# Autodesk Inventor assembly: Assembly1
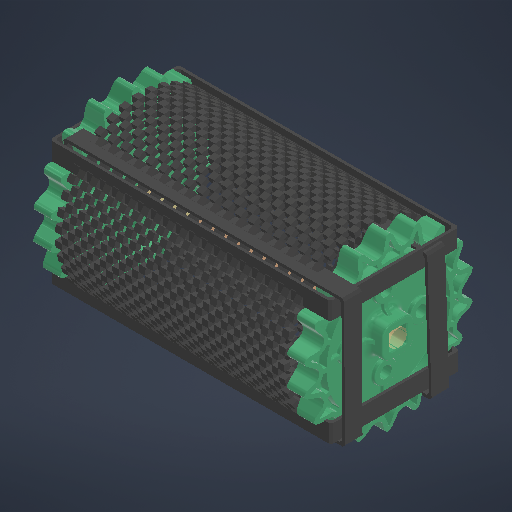
[picture p0: Inventor's stored thumbnail of the model, 512x512]
Saved by Autodesk Inventor 2025.2 (Build 292293000, 293)
## iProperties
Created: 2026-01-02
Part Number: Assembly1
Document SubType Name: Assembly
Designer: cloudy
Author: cloudy
## Documents named in this file (5)
- C:\Users\cloudy\Documents\GitHub\aura-cad\24\Assembly1.iam
- C:\Users\cloudy\Documents\GitHub\aura-cad\24\mesh 2.22.ipt
- C:\Users\cloudy\Documents\GitHub\aura-cad\!lib\Motion\Sprockets\9P Sprocket\9P 18T Sprocket, No Insert.iam
- C:\Users\cloudy\Documents\GitHub\aura-cad\!lib\Motion\Sprockets\9P Sprocket.iam
- C:\Users\cloudy\Documents\GitHub\aura-cad\24\band 18t.ipt
## Components (7 placed, 3 different names)
1. mesh 2.22:1 — Insert:1, Insert:2
2. 9P 18T Sprocket, No Insert:1 [sub-assembly] — Insert:2, Mate:1
3. 9P 18T Sprocket, No Insert:2 [sub-assembly] — Insert:1, Mate:1
4. band 18t:1
5. band 18t:2
6. band 18t:3
7. band 18t:4
## Relationships (3: Insert 2, Mate 1)
- Insert:1: mesh 2.22:1 ↔ 9P 18T Sprocket, No Insert:2
- Insert:2: mesh 2.22:1 ↔ 9P 18T Sprocket, No Insert:1
- Mate:1: 9P 18T Sprocket, No Insert:1 ↔ 9P 18T Sprocket, No Insert:2
